# Autodesk Inventor assembly: CNC_full_assembly
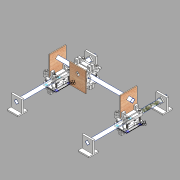
[picture p0: Inventor's stored thumbnail of the model, 180x180]
Saved by Autodesk Inventor 2020 (Build 240168000, 168)
## iProperties
Created: 2021-04-01
Part Number: CNC_full_assembly
Document SubType Name: Assembly
Designer: griss
Author: griss
## Documents named in this file (13)
- C:\Users\griss\Documents\Inventor\CNC\CNC_full_assembly.iam
- C:\Users\griss\Documents\Inventor\CNC\y_axis_carriage\carriage_assemblyiam.iam
- C:\Users\griss\Documents\Inventor\CNC\y_axis_base\base.assembly.iam
- C:\Users\griss\Documents\Inventor\CNC\connections\91309A591_LOW-STRENGTH ZINC-PLATED STEEL CAP SCREW.ipt
- C:\Users\griss\Documents\Inventor\CNC\connections\90473A030_LOW-STRENGTH STEEL HEX NUT.ipt
- C:\Users\griss\Documents\Inventor\CNC\x_axis\x_axis_base_rails.iam
- C:\Users\griss\Documents\Inventor\CNC\y_axis_carriage\universal_carriage_assembly.iam
- C:\Users\griss\Documents\Inventor\CNC\y_axis_carriage\carriage_assembly_top.iam
- C:\Users\griss\Documents\Inventor\CNC\x_axis\x_axis_wood_mount.ipt
- C:\Users\griss\Documents\Inventor\CNC\CNC_full_assembly\AIP\FEA\dkbzbcj40.fins
- C:\Users\griss\Documents\Inventor\CNC\CNC_full_assembly\AIP\FEA\dkbzbcj4w.fsat
- C:\Users\griss\Documents\Inventor\CNC\CNC_full_assembly\AIP\FEA\dkbzbcj4w.ftes
- C:\Users\griss\Documents\Inventor\CNC\CNC_full_assembly\AIP\FEA\dkbzbcj4w.fwiz
## Components (12 placed, 8 different names)
1. 91309A591_LOW-STRENGTH ZINC-PLATED STEEL CAP SCREW:1 — Mate:6, Mate:7, Mate:8
2. 90473A030_LOW-STRENGTH STEEL HEX NUT:1 — Mate:8, Mate:9
3. x_axis_base_rails:1 [sub-assembly] — Mate:10, Mate:11, Flush:2, Tangent:19, Tangent:20, Tangent:21, Tangent:22, Tangent:23, Tangent:24, Tangent:25, Tangent:26
4. universal_carriage_assembly:1 [sub-assembly] — Tangent:11, Tangent:12, Tangent:13, Tangent:14, Flush:3
5. universal_carriage_assembly:2 [sub-assembly] — Flush:4, Tangent:15, Tangent:16, Tangent:17, Tangent:18
6. carriage_assembly_top:1 [sub-assembly] — Tangent:19, Tangent:20, Tangent:21, Tangent:22, Flush:5, Mate:12, Flush:6
7. carriage_assembly_top:2 [sub-assembly] — Tangent:23, Tangent:24, Tangent:25, Tangent:26, Flush:5
8. x_axis_wood_mount:1 — Mate:12, Flush:6
9. carriage_assemblyiam:1 [sub-assembly] — Tangent:1, Tangent:3, Tangent:9, Tangent:10, Mate:6, Mate:7, Mate:9, Mate:10, Mate:11, Flush:2, Flush:3
10. carriage_assemblyiam:2 [sub-assembly] — Flush:4
11. base.assembly:1 [sub-assembly] — Tangent:1, Tangent:3, Tangent:9, Tangent:10, Tangent:11, Tangent:12, Tangent:13, Tangent:14
12. base.assembly:2 [sub-assembly] — Tangent:15, Tangent:16, Tangent:17, Tangent:18
## Component patterns: y axis carriages top (2 elements), y_axis_base (2 elements)
## Relationships (32: Tangent 20, Mate 7, Flush 5)
- Tangent:1: carriage_assemblyiam:1 ↔ base.assembly:1
- Tangent:3: carriage_assemblyiam:1 ↔ base.assembly:1
- Tangent:9: carriage_assemblyiam:1 ↔ base.assembly:1
- Tangent:10: carriage_assemblyiam:1 ↔ base.assembly:1
- Mate:6: 91309A591_LOW-STRENGTH ZINC-PLATED STEEL CAP SCREW:1 ↔ carriage_assemblyiam:1
- Mate:7: 91309A591_LOW-STRENGTH ZINC-PLATED STEEL CAP SCREW:1 ↔ carriage_assemblyiam:1
- Mate:8: 91309A591_LOW-STRENGTH ZINC-PLATED STEEL CAP SCREW:1 ↔ 90473A030_LOW-STRENGTH STEEL HEX NUT:1
- Mate:9: 90473A030_LOW-STRENGTH STEEL HEX NUT:1 ↔ carriage_assemblyiam:1
- Mate:10: x_axis_base_rails:1 ↔ carriage_assemblyiam:1
- Mate:11: x_axis_base_rails:1 ↔ carriage_assemblyiam:1
- Flush:2: x_axis_base_rails:1 ↔ carriage_assemblyiam:1
- Tangent:11: universal_carriage_assembly:1 ↔ base.assembly:1
- Tangent:12: universal_carriage_assembly:1 ↔ base.assembly:1
- Tangent:13: universal_carriage_assembly:1 ↔ base.assembly:1
- Tangent:14: universal_carriage_assembly:1 ↔ base.assembly:1
- Flush:3: universal_carriage_assembly:1 ↔ carriage_assemblyiam:1
- Flush:4: universal_carriage_assembly:2 ↔ carriage_assemblyiam:2
- Tangent:15: universal_carriage_assembly:2 ↔ base.assembly:2
- Tangent:16: universal_carriage_assembly:2 ↔ base.assembly:2
- Tangent:17: universal_carriage_assembly:2 ↔ base.assembly:2
- Tangent:18: universal_carriage_assembly:2 ↔ base.assembly:2
- Tangent:19: x_axis_base_rails:1 ↔ carriage_assembly_top:1
- Tangent:20: x_axis_base_rails:1 ↔ carriage_assembly_top:1
- Tangent:21: x_axis_base_rails:1 ↔ carriage_assembly_top:1
- Tangent:22: x_axis_base_rails:1 ↔ carriage_assembly_top:1
- Tangent:23: x_axis_base_rails:1 ↔ carriage_assembly_top:2
- Tangent:24: x_axis_base_rails:1 ↔ carriage_assembly_top:2
- Tangent:25: x_axis_base_rails:1 ↔ carriage_assembly_top:2
- Tangent:26: x_axis_base_rails:1 ↔ carriage_assembly_top:2
- Flush:5: carriage_assembly_top:1 ↔ carriage_assembly_top:2
- Mate:12: carriage_assembly_top:1 ↔ x_axis_wood_mount:1
- Flush:6: carriage_assembly_top:1 ↔ x_axis_wood_mount:1
## Named parameters: base_width = 609.6 mm, base_length = 304.8 mm, sa_0 = 4448.22
note: some values were not read from the file. Shown as the stored number, unit unknown: "sa_0".
